# Autodesk Inventor assembly: Igus and Arm Bracket_MIR1
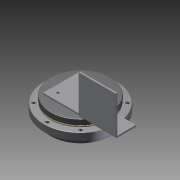
[picture p0: Inventor's stored thumbnail of the model, 180x180]
Saved by Autodesk Inventor 2015 (Build 190159000, 159)
## iProperties
Created: 2015-01-19
Part Number: Igus and Arm Bracket_MIR1
Document SubType Name: Assembly
Designer: chapale16
Author: chapale16
## Documents named in this file (3)
- \\lhssvr02\Homedirs\Robotics Club\CAD Model 2015\Igus and Arm Bracket_MIR1.iam
- \\lhssvr02\Homedirs\Robotics Club\CAD Model 2015\Game Components\The Tote Collector-Arms\Imported Components\PRT_01_30_1\PRT_01_30_1_MIR2.iam
- \\lhssvr02\Homedirs\Robotics Club\CAD Model 2015\Arm holder Bracket_MIR1.ipt
## Components (2 placed, 2 different names)
1. PRT_01_30_1_MIR2:1 [sub-assembly] — Mate:3, Mate:2, Mate:1
2. Arm holder Bracket_MIR1:1 — Mate:3, Mate:2, Mate:1
## Relationships (3: Mate 3)
- Mate:3: PRT_01_30_1_MIR2:1 ↔ Arm holder Bracket_MIR1:1
- Mate:2: PRT_01_30_1_MIR2:1 ↔ Arm holder Bracket_MIR1:1
- Mate:1: PRT_01_30_1_MIR2:1 ↔ Arm holder Bracket_MIR1:1
